# Autodesk Inventor assembly: pancake-direct-v2
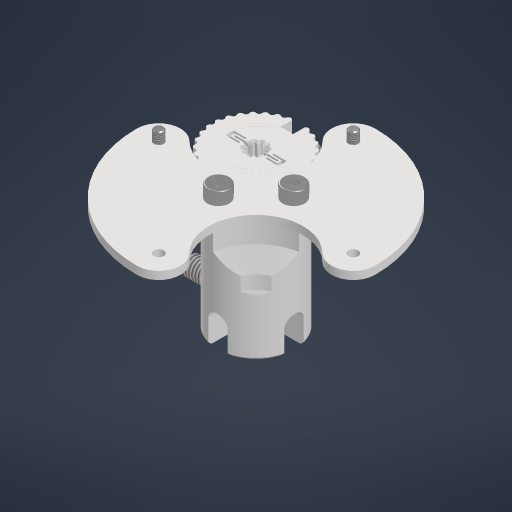
[picture p0: Inventor's stored thumbnail of the model, 512x512]
Saved by Autodesk Inventor 2024 (Build 280153000, 153)
## iProperties
Created: 2024-12-16
Part Number: pancake-direct-v2
Document SubType Name: Assembly
Designer: lokies
Author: lokies
## Documents named in this file (11)
- C:\Users\lokies\Nextcloud\projects\motorized-mounts\mechanical\pancake-direct-v2\pancake-direct-v2.iam
- C:\Users\lokies\Nextcloud\projects\motorized-mounts\mechanical\pancake-direct-v2\mount-plate.ipt
- C:\Users\lokies\Nextcloud\projects\motorized-mounts\mechanical\pancake-direct-v2\gear-grip.ipt
- C:\Users\lokies\Nextcloud\projects\motorized-mounts\mechanical\pancake-direct-v2\screw-grip.ipt
- C:\Users\lokies\Nextcloud\projects\motorized-mounts\mechanical\pancake-direct-v2\fastener.ipt
- C:\Users\lokies\Documents\Inventor\Content Center Files\R2024\en-US\DIN 912\DIN 912 - M2 x 0,4 x 16 x 15.ipt
- C:\Users\lokies\Documents\Inventor\Content Center Files\R2024\en-US\DIN 934\DIN 934 - M2 x 0,4.ipt
- C:\Users\lokies\Nextcloud\projects\motorized-mounts\mechanical\pancake-direct-v2\mount-stem.ipt
- C:\Users\lokies\Documents\Inventor\Content Center Files\R2024\en-US\DIN 912\DIN 912 - M4 x 0,7 x 12 x 10,25.ipt
- C:\Users\lokies\Documents\Inventor\Content Center Files\R2024\en-US\DIN 912\DIN 912 - M3 x 0,5 x 6 x 4,75.ipt
- C:\Users\lokies\Documents\Inventor\Content Center Files\R2024\en-US\DIN 912\DIN 912 - M6 x 1 x 16 x 13,5.ipt
## Components (12 placed, 10 different names)
1. mount-plate:1 — Angle:1, Mate:10, Flush:7, Mate:11, Mate:12, Mate:13, Mate:14, Mate:15, Mate:16, Mate:17, Mate:18, Mate:19
2. gear-grip:1 — Angle:1, Flush:1, Flush:2, Flush:3, Mate:20, Flush:8
3. screw-grip:1 — Flush:1, Flush:2, Flush:3, Flush:4
4. fastener:1 — Flush:4, Mate:6, Mate:7, Mate:8, Mate:9, Angle:2, Mate:20, Flush:8
5. DIN 912 - replaced by DIN EN ISO 4762 M2 x 16:1 — Mate:6, Mate:7
6. DIN 934 - replaced by DIN EN 24032/28673/28674 M2:1 — Mate:8, Mate:9, Angle:2
7. mount-stem:1 — Mate:10, Flush:7, Mate:11, Insert:1
8. DIN 912 - replaced by DIN EN ISO 4762 M4 x 12:1 — Mate:12, Mate:13
9. DIN 912 - replaced by DIN EN ISO 4762 M4 x 12:2 — Mate:14, Mate:15
10. DIN 912 - replaced by DIN EN ISO 4762 M3 x 6:1 — Mate:16, Mate:17
11. DIN 912 - replaced by DIN EN ISO 4762 M3 x 6:2 — Mate:18, Mate:19
12. DIN 912 - replaced by DIN EN ISO 4762 M6 x 16:1 — Insert:1
## Relationships (24: Mate 15, Flush 6, Angle 2, Insert 1)
- Angle:1 (0 deg): mount-plate:1 ↔ gear-grip:1
- Flush:1: gear-grip:1 ↔ screw-grip:1
- Flush:2: gear-grip:1 ↔ screw-grip:1
- Flush:3: gear-grip:1 ↔ screw-grip:1
- Flush:4: screw-grip:1 ↔ fastener:1
- Mate:6: fastener:1 ↔ DIN 912 - replaced by DIN EN ISO 4762 M2 x 16:1
- Mate:7: fastener:1 ↔ DIN 912 - replaced by DIN EN ISO 4762 M2 x 16:1
- Mate:8: fastener:1 ↔ DIN 934 - replaced by DIN EN 24032/28673/28674 M2:1
- Mate:9: fastener:1 ↔ DIN 934 - replaced by DIN EN 24032/28673/28674 M2:1
- Angle:2 (0 deg): fastener:1 ↔ DIN 934 - replaced by DIN EN 24032/28673/28674 M2:1
- Mate:10: mount-plate:1 ↔ mount-stem:1
- Flush:7: mount-plate:1 ↔ mount-stem:1
- Mate:11: mount-plate:1 ↔ mount-stem:1
- Mate:12: mount-plate:1 ↔ DIN 912 - replaced by DIN EN ISO 4762 M4 x 12:1
- Mate:13: mount-plate:1 ↔ DIN 912 - replaced by DIN EN ISO 4762 M4 x 12:1
- Mate:14: mount-plate:1 ↔ DIN 912 - replaced by DIN EN ISO 4762 M4 x 12:2
- Mate:15: mount-plate:1 ↔ DIN 912 - replaced by DIN EN ISO 4762 M4 x 12:2
- Mate:16: mount-plate:1 ↔ DIN 912 - replaced by DIN EN ISO 4762 M3 x 6:1
- Mate:17: mount-plate:1 ↔ DIN 912 - replaced by DIN EN ISO 4762 M3 x 6:1
- Mate:18: mount-plate:1 ↔ DIN 912 - replaced by DIN EN ISO 4762 M3 x 6:2
- Mate:19: mount-plate:1 ↔ DIN 912 - replaced by DIN EN ISO 4762 M3 x 6:2
- Insert:1: mount-stem:1 ↔ DIN 912 - replaced by DIN EN ISO 4762 M6 x 16:1
- Mate:20: gear-grip:1 ↔ fastener:1
- Flush:8: gear-grip:1 ↔ fastener:1
